# Autodesk Inventor assembly: SPE3V1 Freno
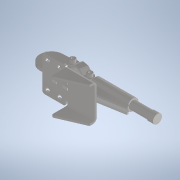
[picture p0: Inventor's stored thumbnail of the model, 180x180]
Saved by Autodesk Inventor 2021.2 (Build 252289000, 289)
## iProperties
Created: 2026-06-23
Part Number: SPE3V1 Freno
Document SubType Name: Assembly
Designer: nelso
Author: nelso
## Documents named in this file (8)
- C:\Users\nelso\Desktop\Soporte-Paciente-Espinografia\Workspace\SPE3V1 Freno.iam
- C:\Users\nelso\Desktop\Soporte-Paciente-Espinografia\Workspace\SP9V1 Columna Freno.ipt
- C:\Users\nelso\Desktop\Soporte-Paciente-Espinografia\Workspace\SP8V1 Conductor Hexagonal Freno.ipt
- C:\Users\nelso\Desktop\Soporte-Paciente-Espinografia\Workspace\SP6V1 Vastago Freno.ipt
- C:\Users\nelso\Desktop\Soporte-Paciente-Espinografia\Workspace\DIN912-M5X0.8L16P.ipt
- C:\Users\nelso\Desktop\Soporte-Paciente-Espinografia\Workspace\SP7V1 Viela Freno.ipt
- C:\Users\nelso\Desktop\Soporte-Paciente-Espinografia\Workspace\DIN555-5M5X0.8C.ipt
- C:\Users\nelso\Desktop\Soporte-Paciente-Espinografia\Workspace\SPE27V1 Soporte Freno.iam
## Components (10 placed, 7 different names)
1. SP9V1 Columna Freno:2 — Flush:4
2. SP8V1 Conductor Hexagonal Freno:1 — Mate:34, Mate:38, Mate:62, Mate:71, Mate:74
3. SP6V1 Vastago Freno:1 — Mate:41, Mate:68
4. DIN912-M5X0.8L16P:1 — Mate:62, Mate:69, Mate:72, Mate:75, Mate:77
5. DIN912-M5X0.8L16P:2 — Mate:68, Mate:70, Mate:73, Mate:76, Mate:80
6. SP7V1 Viela Freno:1 — Mate:69, Mate:70, Mate:71, Mate:78, Mate:79
7. SP7V1 Viela Freno:2 — Mate:72, Mate:73, Mate:74, Mate:75, Mate:76
8. DIN555-5M5X0.8C:1 — Mate:77, Mate:78
9. DIN555-5M5X0.8C:2 — Mate:79, Mate:80
10. SPE5V1 Soporte Freno:1 [sub-assembly]
## Relationships (29: Mate 24, Flush 4, Tangent 1)
- [Mate]: SPE5V1 Soporte Freno:1
- [Flush]: SPE5V1 Soporte Freno:1
- [Mate]: SP9V1 Columna Freno:2 ↔ SPE5V1 Soporte Freno:1
- [Mate]: SPE5V1 Soporte Freno:1
- Mate:34: SP8V1 Conductor Hexagonal Freno:1
- [Flush] (4 mm): SPE5V1 Soporte Freno:1
- [Mate]: SPE5V1 Soporte Freno:1
- Flush:4 (-4 mm): SP9V1 Columna Freno:2
- Mate:38: SP8V1 Conductor Hexagonal Freno:1
- [Mate]: SPE5V1 Soporte Freno:1
- [Tangent]: SP9V1 Columna Freno:2 ↔ SPE5V1 Soporte Freno:1
- Mate:41: SP6V1 Vastago Freno:1
- [Mate]: SP6V1 Vastago Freno:1 ↔ SPE5V1 Soporte Freno:1
- [Flush] (-18 mm): SP6V1 Vastago Freno:1 ↔ SPE5V1 Soporte Freno:1
- [Mate]: SP9V1 Columna Freno:2 ↔ SPE5V1 Soporte Freno:1
- Mate:62: SP8V1 Conductor Hexagonal Freno:1 ↔ DIN912-M5X0.8L16P:1
- Mate:68: SP6V1 Vastago Freno:1 ↔ DIN912-M5X0.8L16P:2
- Mate:69: DIN912-M5X0.8L16P:1 ↔ SP7V1 Viela Freno:1
- Mate:70: DIN912-M5X0.8L16P:2 ↔ SP7V1 Viela Freno:1
- Mate:71: SP8V1 Conductor Hexagonal Freno:1 ↔ SP7V1 Viela Freno:1
- Mate:72: DIN912-M5X0.8L16P:1 ↔ SP7V1 Viela Freno:2
- Mate:73: DIN912-M5X0.8L16P:2 ↔ SP7V1 Viela Freno:2
- Mate:74: SP8V1 Conductor Hexagonal Freno:1 ↔ SP7V1 Viela Freno:2
- Mate:75: DIN912-M5X0.8L16P:1 ↔ SP7V1 Viela Freno:2
- Mate:76: DIN912-M5X0.8L16P:2 ↔ SP7V1 Viela Freno:2
- Mate:77: DIN912-M5X0.8L16P:1 ↔ DIN555-5M5X0.8C:1
- Mate:78: SP7V1 Viela Freno:1 ↔ DIN555-5M5X0.8C:1
- Mate:79: SP7V1 Viela Freno:1 ↔ DIN555-5M5X0.8C:2
- Mate:80: DIN912-M5X0.8L16P:2 ↔ DIN555-5M5X0.8C:2
